# Autodesk Inventor assembly: Test Assembly - small
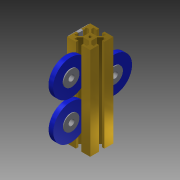
[picture p0: Inventor's stored thumbnail of the model, 180x180]
Saved by Autodesk Inventor 2014 (Build 180170000, 170)
## iProperties
Created: 2015-02-07
Part Number: Test Assembly - small
Document SubType Name: Assembly
Designer: Spooner
Author: Spooner
## Documents named in this file (5)
- C:\Users\Spooner\Documents\Inventor\80-20  Linear Bearing\Test Assembly - small.iam
- C:\Users\Spooner\Documents\Inventor\80-20  Linear Bearing\1_5 80-20 x 6in.ipt
- C:\Users\Spooner\Documents\Inventor\80-20  Linear Bearing\Small Bearing.ipt
- C:\Users\Spooner\Documents\Inventor\80-20  Linear Bearing\Small Bearing Cover.ipt
- C:\Users\Spooner\Documents\Inventor\80-20  Linear Bearing\Flat Bearing.ipt
## Components (8 placed, 4 different names)
1. 1_5 80-20 x 6in:1 — Mate:1, Mate:2, Mate:3, Mate:5, Mate:6, Flush:4, Flush:5
2. Small Bearing:1 — Mate:1, Mate:4, Mate:7, Insert:1, Flush:3
3. Small Bearing:2 — Mate:2, Mate:4, Mate:5, Mate:7, Flush:2, Mate:8
4. Small Bearing:3 — Mate:3, Mate:6, Insert:2, Flush:3
5. Small Bearing Cover:1 — Flush:2, Mate:8
6. Small Bearing Cover:2 — Insert:2
7. Small Bearing Cover:3 — Insert:1
8. Flat Bearing:1 — Flush:4, Flush:5
## Relationships (14: Mate 8, Flush 4, Insert 2)
- Mate:1: 1_5 80-20 x 6in:1 ↔ Small Bearing:1
- Mate:2: 1_5 80-20 x 6in:1 ↔ Small Bearing:2
- Mate:3: 1_5 80-20 x 6in:1 ↔ Small Bearing:3
- Mate:4: Small Bearing:1 ↔ Small Bearing:2
- Mate:5 (16.8275 mm): 1_5 80-20 x 6in:1 ↔ Small Bearing:2
- Mate:6 (16.8275 mm): 1_5 80-20 x 6in:1 ↔ Small Bearing:3
- Mate:7 (-63.5 mm): Small Bearing:1 ↔ Small Bearing:2
- Flush:2: Small Bearing:2 ↔ Small Bearing Cover:1
- Mate:8: Small Bearing:2 ↔ Small Bearing Cover:1
- Insert:1: Small Bearing:1 ↔ Small Bearing Cover:3
- Insert:2: Small Bearing:3 ↔ Small Bearing Cover:2
- Flush:3 (31.75 mm): Small Bearing:1 ↔ Small Bearing:3
- Flush:4: 1_5 80-20 x 6in:1 ↔ Flat Bearing:1
- Flush:5: 1_5 80-20 x 6in:1 ↔ Flat Bearing:1
